# Autodesk Inventor assembly: Drivetrain Side
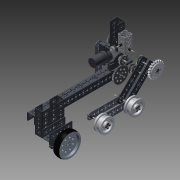
[picture p0: Inventor's stored thumbnail of the model, 180x180]
Saved by Autodesk Inventor 2015 (Build 190159000, 159)
## iProperties
Created: 2015-09-28
Part Number: Drivetrain Side
Document SubType Name: Assembly
Designer: Jing-Chen
Author: Jing-Chen
## Documents named in this file (25)
- C:\Users\Jing-Chen\Desktop\Bionic Hybrids 2016\Bionic-Hybrids\CAD\Drivetrain\Sub-Assemblies\Drivetrain Side.iam
- C:\Users\Jing-Chen\Desktop\Bionic Hybrids 2016\Bionic-Hybrids\Stock\Bracket-U25 - 739069.ipt
- C:\Users\Jing-Chen\Desktop\Bionic Hybrids 2016\Bionic-Hybrids\CAD\Drivetrain\Sub-Assemblies\Wheel Assembly.iam
- C:\Users\Jing-Chen\Desktop\Bionic Hybrids 2016\Bionic-Hybrids\CAD\Drivetrain\Sub-Assemblies\Track Frame Assembly.iam
- C:\Users\Jing-Chen\Desktop\Bionic Hybrids 2016\Bionic-Hybrids\Stock\Bearing-Thrust - 739091.ipt
- C:\Users\Jing-Chen\Desktop\Bionic Hybrids 2016\Bionic-Hybrids\Stock\Motor Mount - 739089.ipt
- C:\Users\Jing-Chen\Desktop\Bionic Hybrids 2016\Bionic-Hybrids\Stock\Bracket-U5 - 739066.ipt
- C:\Users\Jing-Chen\Desktop\Bionic Hybrids 2016\Bionic-Hybrids\CAD\General\Modified Parts\Movable Motor.iam
- C:\Users\Jing-Chen\Desktop\Bionic Hybrids 2016\Bionic-Hybrids\Stock\Gear-80 tooth - 731901.ipt
- C:\Users\Jing-Chen\Desktop\Bionic Hybrids 2016\Bionic-Hybrids\Stock\Plate-2x1 Long - 739061.ipt
- C:\Users\Jing-Chen\Desktop\Bionic Hybrids 2016\Bionic-Hybrids\Stock\Shaft Collar-Setscrew, Axle, Mountable - 739079.iam
- C:\Users\Jing-Chen\Desktop\Bionic Hybrids 2016\Bionic-Hybrids\Stock\Screw 0.5in - 739097.ipt
- C:\Users\Jing-Chen\Desktop\Bionic Hybrids 2016\Bionic-Hybrids\Stock\Shaft Collar-Setscrew, Axle, Mountable - 739172.iam
- C:\Users\Jing-Chen\Desktop\Bionic Hybrids 2016\Bionic-Hybrids\Stock\Gear-40 tooth - 731901.ipt
- C:\Users\Jing-Chen\Desktop\Bionic Hybrids 2016\Bionic-Hybrids\Stock\Nut-Locking - 739094.ipt
- C:\Users\Jing-Chen\Desktop\Bionic Hybrids 2016\Bionic-Hybrids\CAD\General\40-tooth Gear Assembly.iam
- C:\Users\Jing-Chen\Desktop\Bionic Hybrids 2016\Bionic-Hybrids\Stock\Plate-9x1 - 739272.ipt
- C:\Users\Jing-Chen\Desktop\Bionic Hybrids 2016\Bionic-Hybrids\New Stock\Worm Gear Abstract.iam
- C:\Users\Jing-Chen\Desktop\Bionic Hybrids 2016\Bionic-Hybrids\Stock\Shaft Collar-Setscrew, Axle - 739092.iam
- C:\Users\Jing-Chen\Desktop\Bionic Hybrids 2016\Bionic-Hybrids\CAD\General\Modified Parts\55mm axle.ipt
- C:\Users\Jing-Chen\Desktop\Bionic Hybrids 2016\Bionic-Hybrids\Stock\Axle-100mm - 739088.ipt
- C:\Users\Jing-Chen\Desktop\Bionic Hybrids 2016\Bionic-Hybrids\CAD\General\Modified Parts\Cut 100mm axle.ipt
- C:\Users\Jing-Chen\Desktop\Bionic Hybrids 2016\Bionic-Hybrids\Stock\Screw 1.5in - 739195.ipt
- C:\Users\Jing-Chen\Desktop\Bionic Hybrids 2016\Bionic-Hybrids\Stock\Bracket-U9 - 739067.ipt
- C:\Users\Jing-Chen\Desktop\Bionic Hybrids 2016\Bionic-Hybrids\CAD\Drivetrain\Sub-Assemblies\Track Frame Assembly with Side Guards.iam
## Components (77 placed, 24 different names)
1. Track Frame Assembly:1 [sub-assembly] — Mate:33, Mate:36, Rotation:2, Mate:157, Mate:160, Angle:11, Mate:258, Mate:259, Flush:11
2. Bearing-Thrust - 739091:1 — Mate:33, Mate:36, Mate:60, Mate:61
3. Motor Mount - 739089:1 — Mate:40, Flush:1, Mate:51, Mate:52, Mate:53, Mate:234, Mate:235, Mate:236, Mate:237
4. Wheel Assembly:1 [sub-assembly] — Angle:2, Mate:41, Flush:2
5. Movable Motor:1 [sub-assembly] — Mate:40, Flush:1, Angle:1, Angle:2, Mate:41, Flush:2
6. Bracket-U5 - 739066:1 — Mate:44, Mate:46, Mate:47, Mate:51, Mate:52, Mate:53, Mate:248, Mate:249
7. Bracket-U5 - 739066:2 — Mate:44, Mate:46, Mate:47, Mate:54, Mate:55, Mate:56
8. Bracket-U5 - 739066:3 — Mate:57, Mate:58, Mate:59
9. Bracket-U25 - 739069:1 — Mate:54, Mate:55, Mate:56, Mate:57, Mate:58, Mate:59, Mate:60, Mate:61, Mate:62, Angle:3, Mate:81, Mate:96, Mate:97, Mate:126, Mate:128, Mate:130, Mate:131, Mate:132, Mate:133, Mate:135, Mate:137, Mate:140, Mate:141, Mate:165, Mate:170, Mate:173, Mate:198, Mate:204, Mate:212, Mate:230, Mate:233
10. Movable Motor:2 [sub-assembly] — Mate:64, Flush:3, Angle:4, Angle:5, Mate:108
11. Motor Mount - 739089:2 — Mate:62, Angle:3, Mate:64, Flush:3, Mate:82, Mate:83, Mate:116, Mate:199, Mate:200, Mate:202, Mate:203
12. Plate-2x1 Long - 739061:2 — Mate:81, Mate:82, Mate:83, Mate:116
13. Shaft Collar-Setscrew, Axle, Mountable - 739079:1 [sub-assembly] — Angle:5, Mate:104, Mate:105, Mate:106, Mate:107, Mate:108, Mate:109, Mate:111
14. Screw 0.5in - 739097:1 — Mate:105, Mate:110, Mate:113
15. Screw 0.5in - 739097:2 — Mate:107, Mate:112
16. Screw 0.5in - 739097:3 — Mate:104, Mate:114
17. Screw 0.5in - 739097:4 — Mate:106, Mate:115
18. Bearing-Thrust - 739091:2 — Mate:96, Mate:97, Mate:100
19. Shaft Collar-Setscrew, Axle, Mountable - 739172:1 [sub-assembly] — Mate:100, Mate:102, Mate:103, Mate:121, Mate:122, Mate:123, Mate:124, Mate:179
20. Gear-80 tooth - 731901:2 — Mate:102, Mate:103, Flush:4, Rotation:1, Rotation:2, Mate:117, Mate:118, Mate:119, Mate:120, Mate:178, Flush:7
21. Gear-40 tooth - 731901:1 — Mate:109, Mate:110, Mate:111, Mate:112, Mate:113, Mate:114, Mate:115, Flush:4, Rotation:1
22. Screw 0.5in - 739097:5 — Mate:118, Mate:122
23. Screw 0.5in - 739097:6 — Mate:117, Mate:121
24. Screw 0.5in - 739097:7 — Mate:119, Mate:123
25. Screw 0.5in - 739097:8 — Mate:120, Mate:124, Mate:178
26. Bearing-Thrust - 739091:3 — Mate:126, Mate:128, Mate:177, Mate:181
27. Screw 0.5in - 739097:9 — Mate:133, Mate:134, Mate:207, Mate:208
28. Screw 0.5in - 739097:10 — Mate:131, Mate:136, Mate:206, Mate:209
29. Screw 0.5in - 739097:11 — Mate:130, Mate:139, Mate:210
30. Screw 0.5in - 739097:12 — Mate:132, Mate:138, Mate:211
31. Nut-Locking - 739094:1 — Mate:136, Mate:137
32. Nut-Locking - 739094:2 — Mate:134, Mate:135
33. Nut-Locking - 739094:3 — Mate:139, Mate:140
34. Nut-Locking - 739094:4 — Mate:138, Mate:141
35. Bearing-Thrust - 739091:4 — Mate:158, Mate:160, Mate:221
36. Bearing-Thrust - 739091:5 — Mate:182, Mate:184, Mate:219, Mate:220
37. Bearing-Thrust - 739091:6 — Mate:187, Mate:189, Mate:215, Mate:216
38. Bearing-Thrust - 739091:7 — Mate:186, Mate:217, Mate:218
39. 40-tooth Gear Assembly:1 [sub-assembly] — Mate:157, Mate:158, Angle:11, Rotation:4
40. 40-tooth Gear Assembly:2 [sub-assembly] — Mate:183, Mate:184, Flush:8, Rotation:3, Rotation:4
41. 40-tooth Gear Assembly:3 [sub-assembly] — Mate:188, Mate:189, Flush:9, Rotation:3, Angle:14
42. Movable Motor:3 [sub-assembly] — Mate:169, Flush:6, Angle:7, Angle:12, Mate:191, Flush:10, Mate:192
43. Motor Mount - 739089:3 — Mate:169, Flush:6, Mate:171, Angle:10, Mate:172, Mate:238, Mate:239, Mate:240, Mate:241
44. Plate-9x1 - 739272:1 — Mate:165, Mate:170, Mate:171, Angle:10, Mate:172, Mate:173, Mate:226, Mate:227, Mate:228, Mate:229, Mate:243, Mate:247
45. Worm Gearbox, Ratio 20:1 [sub-assembly] — Mate:190, Mate:213, Mate:214, Mate:224
46. 55mm axle:1 — Mate:177, Mate:179, Flush:7, Mate:180
47. Shaft Collar-Setscrew, Axle - 739092:1 [sub-assembly] — Mate:180, Mate:181
48. Shaft Collar-Setscrew, Axle - 739092:2 [sub-assembly] — Mate:185, Mate:186
49. 55mm axle:2 — Mate:182, Mate:183, Flush:8, Mate:185
50. Axle-100mm - 739088:1 — Mate:187, Mate:188, Flush:9, Rotation:5, Angle:14, Mate:214
51. Shaft Collar-Setscrew, Axle, Mountable - 739079:2 [sub-assembly] — Angle:12, Mate:191, Flush:10, Mate:194, Mate:195
52. Shaft Collar-Setscrew, Axle, Mountable - 739172:2 [sub-assembly] — Angle:13, Mate:193, Mate:194, Mate:195, Mate:250, Mate:251, Mate:252, Mate:253, Mate:254, Mate:255, Mate:256, Mate:257
53. Cut 100mm axle:1 — Mate:190, Mate:192, Angle:13, Mate:193, Rotation:5
54. Screw 1.5in - 739195:1 — Mate:199, Mate:200, Mate:201
55. Screw 0.5in - 739097:22 — Mate:222, Mate:223, Mate:225
56. Screw 0.5in - 739097:23 — Mate:227, Mate:229, Mate:232
57. Nut-Locking - 739094:5 — Mate:223, Mate:224
58. Nut-Locking - 739094:6 — Mate:230, Mate:231
59. Nut-Locking - 739094:7 — Mate:198, Mate:201
60. Nut-Locking - 739094:8 — Mate:204, Mate:205
61. Screw 0.5in - 739097:24 — Mate:226, Mate:228, Mate:231
62. Screw 1.5in - 739195:2 — Mate:202, Mate:203, Mate:205
63. Bracket-U9 - 739067:1 — Mate:206, Mate:207, Mate:208, Mate:209, Mate:210, Mate:211, Mate:212, Mate:213, Mate:215, Mate:216, Mate:217, Mate:218, Mate:219, Mate:220, Mate:221, Mate:222, Mate:225
64. Nut-Locking - 739094:9 — Mate:232, Mate:233
65. Screw 1.5in - 739195:3 — Mate:236, Mate:237, Mate:244
66. Screw 1.5in - 739195:4 — Mate:238, Mate:239, Mate:242
67. Screw 1.5in - 739195:5 — Mate:234, Mate:235, Mate:245
68. Screw 1.5in - 739195:6 — Mate:240, Mate:241, Mate:246
69. Nut-Locking - 739094:10 — Mate:242, Mate:243
70. Nut-Locking - 739094:11 — Mate:244, Mate:249
71. Nut-Locking - 739094:12 — Mate:245, Mate:248
72. Nut-Locking - 739094:13 — Mate:246, Mate:247
73. Screw 0.5in - 739097:25 — Mate:255, Mate:257
74. Screw 0.5in - 739097:26 — Mate:254, Mate:256
75. Screw 0.5in - 739097:27 — Mate:251, Mate:252
76. Screw 0.5in - 739097:28 — Mate:250, Mate:253
77. Track Frame Assembly with Side Guards:1 [sub-assembly] — Mate:258, Mate:259, Flush:11
## Relationships (179: Mate 153, Angle 11, Flush 10, RelateRotation 5)
- Mate:33: Track Frame Assembly:1 ↔ Bearing-Thrust - 739091:1
- Mate:36: Track Frame Assembly:1 ↔ Bearing-Thrust - 739091:1
- Mate:40: Motor Mount - 739089:1 ↔ Movable Motor:1
- Flush:1: Motor Mount - 739089:1 ↔ Movable Motor:1
- Angle:1 (180 deg): Movable Motor:1
- Angle:2 (180 deg): Wheel Assembly:1 ↔ Movable Motor:1
- Mate:41: Wheel Assembly:1 ↔ Movable Motor:1
- Flush:2: Wheel Assembly:1 ↔ Movable Motor:1
- Mate:44: Bracket-U5 - 739066:1 ↔ Bracket-U5 - 739066:2
- Mate:46: Bracket-U5 - 739066:1 ↔ Bracket-U5 - 739066:2
- Mate:47: Bracket-U5 - 739066:1 ↔ Bracket-U5 - 739066:2
- Mate:51: Motor Mount - 739089:1 ↔ Bracket-U5 - 739066:1
- Mate:52: Motor Mount - 739089:1 ↔ Bracket-U5 - 739066:1
- Mate:53: Motor Mount - 739089:1 ↔ Bracket-U5 - 739066:1
- Mate:54: Bracket-U5 - 739066:2 ↔ Bracket-U25 - 739069:1
- Mate:55: Bracket-U5 - 739066:2 ↔ Bracket-U25 - 739069:1
- Mate:56: Bracket-U5 - 739066:2 ↔ Bracket-U25 - 739069:1
- Mate:57: Bracket-U5 - 739066:3 ↔ Bracket-U25 - 739069:1
- Mate:58: Bracket-U5 - 739066:3 ↔ Bracket-U25 - 739069:1
- Mate:59: Bracket-U5 - 739066:3 ↔ Bracket-U25 - 739069:1
- Mate:60: Bearing-Thrust - 739091:1 ↔ Bracket-U25 - 739069:1
- Mate:61: Bearing-Thrust - 739091:1 ↔ Bracket-U25 - 739069:1
- Mate:62: Bracket-U25 - 739069:1 ↔ Motor Mount - 739089:2
- Angle:3 (0 deg): Bracket-U25 - 739069:1 ↔ Motor Mount - 739089:2
- Mate:64: Movable Motor:2 ↔ Motor Mount - 739089:2
- Flush:3: Movable Motor:2 ↔ Motor Mount - 739089:2
- Angle:4 (190 deg): Movable Motor:2
- Mate:81: Bracket-U25 - 739069:1 ↔ Plate-2x1 Long - 739061:2
- Mate:82: Motor Mount - 739089:2 ↔ Plate-2x1 Long - 739061:2
- Mate:83: Motor Mount - 739089:2 ↔ Plate-2x1 Long - 739061:2
- Angle:5 (180 deg): Movable Motor:2 ↔ Shaft Collar-Setscrew, Axle, Mountable - 739079:1
- Mate:96: Bracket-U25 - 739069:1 ↔ Bearing-Thrust - 739091:2
- Mate:97: Bracket-U25 - 739069:1 ↔ Bearing-Thrust - 739091:2
- Mate:100: Bearing-Thrust - 739091:2 ↔ Shaft Collar-Setscrew, Axle, Mountable - 739172:1
- Mate:102: Shaft Collar-Setscrew, Axle, Mountable - 739172:1 ↔ Gear-80 tooth - 731901:2
- Mate:103: Shaft Collar-Setscrew, Axle, Mountable - 739172:1 ↔ Gear-80 tooth - 731901:2
- Mate:104: Shaft Collar-Setscrew, Axle, Mountable - 739079:1 ↔ Screw 0.5in - 739097:3
- Mate:105: Shaft Collar-Setscrew, Axle, Mountable - 739079:1 ↔ Screw 0.5in - 739097:1
- Mate:106: Shaft Collar-Setscrew, Axle, Mountable - 739079:1 ↔ Screw 0.5in - 739097:4
- Mate:107: Shaft Collar-Setscrew, Axle, Mountable - 739079:1 ↔ Screw 0.5in - 739097:2
- Mate:108: Movable Motor:2 ↔ Shaft Collar-Setscrew, Axle, Mountable - 739079:1
- Mate:109: Shaft Collar-Setscrew, Axle, Mountable - 739079:1 ↔ Gear-40 tooth - 731901:1
- Mate:110: Screw 0.5in - 739097:1 ↔ Gear-40 tooth - 731901:1
- Mate:111: Shaft Collar-Setscrew, Axle, Mountable - 739079:1 ↔ Gear-40 tooth - 731901:1
- Mate:112: Screw 0.5in - 739097:2 ↔ Gear-40 tooth - 731901:1
- Mate:113: Screw 0.5in - 739097:1 ↔ Gear-40 tooth - 731901:1
- Mate:114: Screw 0.5in - 739097:3 ↔ Gear-40 tooth - 731901:1
- Mate:115: Screw 0.5in - 739097:4 ↔ Gear-40 tooth - 731901:1
- Mate:116: Motor Mount - 739089:2 ↔ Plate-2x1 Long - 739061:2
- Flush:4: Gear-80 tooth - 731901:2 ↔ Gear-40 tooth - 731901:1
- Rotation:1 [RelateRotation] (0.5 ul): Gear-80 tooth - 731901:2 ↔ Gear-40 tooth - 731901:1
- Rotation:2 [RelateRotation] (2 ul): Track Frame Assembly:1 ↔ Gear-80 tooth - 731901:2
- Mate:117: Gear-80 tooth - 731901:2 ↔ Screw 0.5in - 739097:6
- Mate:118: Gear-80 tooth - 731901:2 ↔ Screw 0.5in - 739097:5
- Mate:119: Gear-80 tooth - 731901:2 ↔ Screw 0.5in - 739097:7
- Mate:120: Gear-80 tooth - 731901:2 ↔ Screw 0.5in - 739097:8
- Mate:121: Shaft Collar-Setscrew, Axle, Mountable - 739172:1 ↔ Screw 0.5in - 739097:6
- Mate:122: Shaft Collar-Setscrew, Axle, Mountable - 739172:1 ↔ Screw 0.5in - 739097:5
- Mate:123: Shaft Collar-Setscrew, Axle, Mountable - 739172:1 ↔ Screw 0.5in - 739097:7
- Mate:124: Shaft Collar-Setscrew, Axle, Mountable - 739172:1 ↔ Screw 0.5in - 739097:8
- Mate:126: Bracket-U25 - 739069:1 ↔ Bearing-Thrust - 739091:3
- Mate:128: Bracket-U25 - 739069:1 ↔ Bearing-Thrust - 739091:3
- Mate:130: Bracket-U25 - 739069:1 ↔ Screw 0.5in - 739097:11
- Mate:131: Bracket-U25 - 739069:1 ↔ Screw 0.5in - 739097:10
- Mate:132: Bracket-U25 - 739069:1 ↔ Screw 0.5in - 739097:12
- Mate:133: Bracket-U25 - 739069:1 ↔ Screw 0.5in - 739097:9
- Mate:134: Screw 0.5in - 739097:9 ↔ Nut-Locking - 739094:2
- Mate:135: Bracket-U25 - 739069:1 ↔ Nut-Locking - 739094:2
- Mate:136: Screw 0.5in - 739097:10 ↔ Nut-Locking - 739094:1
- Mate:137: Bracket-U25 - 739069:1 ↔ Nut-Locking - 739094:1
- Mate:138: Screw 0.5in - 739097:12 ↔ Nut-Locking - 739094:4
- Mate:139: Screw 0.5in - 739097:11 ↔ Nut-Locking - 739094:3
- Mate:140: Bracket-U25 - 739069:1 ↔ Nut-Locking - 739094:3
- Mate:141: Bracket-U25 - 739069:1 ↔ Nut-Locking - 739094:4
- Mate:157: Track Frame Assembly:1 ↔ 40-tooth Gear Assembly:1
- Mate:158: Bearing-Thrust - 739091:4 ↔ 40-tooth Gear Assembly:1
- Mate:160: Track Frame Assembly:1 ↔ Bearing-Thrust - 739091:4
- Mate:165: Bracket-U25 - 739069:1 ↔ Plate-9x1 - 739272:1
- Mate:169: Movable Motor:3 ↔ Motor Mount - 739089:3
- Flush:6: Movable Motor:3 ↔ Motor Mount - 739089:3
- Angle:7 (180 deg): Movable Motor:3
- Mate:170: Bracket-U25 - 739069:1 ↔ Plate-9x1 - 739272:1
- Mate:171: Motor Mount - 739089:3 ↔ Plate-9x1 - 739272:1
- Angle:10 (180 deg): Motor Mount - 739089:3 ↔ Plate-9x1 - 739272:1
- Mate:172: Motor Mount - 739089:3 ↔ Plate-9x1 - 739272:1
- Mate:173: Bracket-U25 - 739069:1 ↔ Plate-9x1 - 739272:1
- Mate:177: Bearing-Thrust - 739091:3 ↔ 55mm axle:1
- Mate:178: Gear-80 tooth - 731901:2 ↔ Screw 0.5in - 739097:8
- Mate:179: Shaft Collar-Setscrew, Axle, Mountable - 739172:1 ↔ 55mm axle:1
- Flush:7: Gear-80 tooth - 731901:2 ↔ 55mm axle:1
- Mate:180: 55mm axle:1 ↔ Shaft Collar-Setscrew, Axle - 739092:1
- Mate:181: Bearing-Thrust - 739091:3 ↔ Shaft Collar-Setscrew, Axle - 739092:1
- Mate:182: Bearing-Thrust - 739091:5 ↔ 55mm axle:2
- Mate:183: 40-tooth Gear Assembly:2 ↔ 55mm axle:2
- Mate:184: Bearing-Thrust - 739091:5 ↔ 40-tooth Gear Assembly:2
- Flush:8: 40-tooth Gear Assembly:2 ↔ 55mm axle:2
- Angle:11 (180 deg): Track Frame Assembly:1 ↔ 40-tooth Gear Assembly:1
- Mate:185: Shaft Collar-Setscrew, Axle - 739092:2 ↔ 55mm axle:2
- Mate:186: Bearing-Thrust - 739091:7 ↔ Shaft Collar-Setscrew, Axle - 739092:2
- Mate:187: Bearing-Thrust - 739091:6 ↔ Axle-100mm - 739088:1
- Mate:188: 40-tooth Gear Assembly:3 ↔ Axle-100mm - 739088:1
- Mate:189: Bearing-Thrust - 739091:6 ↔ 40-tooth Gear Assembly:3
- Flush:9: 40-tooth Gear Assembly:3 ↔ Axle-100mm - 739088:1
- Rotation:3 [RelateRotation] (1 ul): 40-tooth Gear Assembly:2 ↔ 40-tooth Gear Assembly:3
- Rotation:4 [RelateRotation] (1 ul): 40-tooth Gear Assembly:1 ↔ 40-tooth Gear Assembly:2
- Mate:190: Worm Gearbox, Ratio 20:1 ↔ Cut 100mm axle:1
- Angle:12 (180 deg): Movable Motor:3 ↔ Shaft Collar-Setscrew, Axle, Mountable - 739079:2
- Mate:191: Movable Motor:3 ↔ Shaft Collar-Setscrew, Axle, Mountable - 739079:2
- Flush:10: Movable Motor:3 ↔ Shaft Collar-Setscrew, Axle, Mountable - 739079:2
- Mate:192: Movable Motor:3 ↔ Cut 100mm axle:1
- Angle:13 (180 deg): Shaft Collar-Setscrew, Axle, Mountable - 739172:2 ↔ Cut 100mm axle:1
- Mate:193: Shaft Collar-Setscrew, Axle, Mountable - 739172:2 ↔ Cut 100mm axle:1
- Mate:194: Shaft Collar-Setscrew, Axle, Mountable - 739079:2 ↔ Shaft Collar-Setscrew, Axle, Mountable - 739172:2
- Mate:195: Shaft Collar-Setscrew, Axle, Mountable - 739079:2 ↔ Shaft Collar-Setscrew, Axle, Mountable - 739172:2
- Rotation:5 [RelateRotation] (0.05 ul): Axle-100mm - 739088:1 ↔ Cut 100mm axle:1
- Angle:14 (180 deg): 40-tooth Gear Assembly:3 ↔ Axle-100mm - 739088:1
- Mate:198: Bracket-U25 - 739069:1 ↔ Nut-Locking - 739094:7
- Mate:199: Motor Mount - 739089:2 ↔ Screw 1.5in - 739195:1
- Mate:200: Motor Mount - 739089:2 ↔ Screw 1.5in - 739195:1
- Mate:201: Screw 1.5in - 739195:1 ↔ Nut-Locking - 739094:7
- Mate:202: Motor Mount - 739089:2 ↔ Screw 1.5in - 739195:2
- Mate:203: Motor Mount - 739089:2 ↔ Screw 1.5in - 739195:2
- Mate:204: Bracket-U25 - 739069:1 ↔ Nut-Locking - 739094:8
- Mate:205: Nut-Locking - 739094:8 ↔ Screw 1.5in - 739195:2
- Mate:206: Screw 0.5in - 739097:10 ↔ Bracket-U9 - 739067:1
- Mate:207: Screw 0.5in - 739097:9 ↔ Bracket-U9 - 739067:1
- Mate:208: Screw 0.5in - 739097:9 ↔ Bracket-U9 - 739067:1
- Mate:209: Screw 0.5in - 739097:10 ↔ Bracket-U9 - 739067:1
- Mate:210: Screw 0.5in - 739097:11 ↔ Bracket-U9 - 739067:1
- Mate:211: Screw 0.5in - 739097:12 ↔ Bracket-U9 - 739067:1
- Mate:212: Bracket-U25 - 739069:1 ↔ Bracket-U9 - 739067:1
- Mate:213: Worm Gearbox, Ratio 20:1 ↔ Bracket-U9 - 739067:1
- Mate:214: Worm Gearbox, Ratio 20:1 ↔ Axle-100mm - 739088:1
- Mate:215: Bearing-Thrust - 739091:6 ↔ Bracket-U9 - 739067:1
- Mate:216: Bearing-Thrust - 739091:6 ↔ Bracket-U9 - 739067:1
- Mate:217: Bearing-Thrust - 739091:7 ↔ Bracket-U9 - 739067:1
- Mate:218: Bearing-Thrust - 739091:7 ↔ Bracket-U9 - 739067:1
- Mate:219: Bearing-Thrust - 739091:5 ↔ Bracket-U9 - 739067:1
- Mate:220: Bearing-Thrust - 739091:5 ↔ Bracket-U9 - 739067:1
- Mate:221: Bearing-Thrust - 739091:4 ↔ Bracket-U9 - 739067:1
- Mate:222: Screw 0.5in - 739097:22 ↔ Bracket-U9 - 739067:1
- Mate:223: Screw 0.5in - 739097:22 ↔ Nut-Locking - 739094:5
- Mate:224: Worm Gearbox, Ratio 20:1 ↔ Nut-Locking - 739094:5
- Mate:225: Screw 0.5in - 739097:22 ↔ Bracket-U9 - 739067:1
- Mate:226: Plate-9x1 - 739272:1 ↔ Screw 0.5in - 739097:24
- Mate:227: Plate-9x1 - 739272:1 ↔ Screw 0.5in - 739097:23
- Mate:228: Plate-9x1 - 739272:1 ↔ Screw 0.5in - 739097:24
- Mate:229: Plate-9x1 - 739272:1 ↔ Screw 0.5in - 739097:23
- Mate:230: Bracket-U25 - 739069:1 ↔ Nut-Locking - 739094:6
- Mate:231: Nut-Locking - 739094:6 ↔ Screw 0.5in - 739097:24
- Mate:232: Screw 0.5in - 739097:23 ↔ Nut-Locking - 739094:9
- Mate:233: Bracket-U25 - 739069:1 ↔ Nut-Locking - 739094:9
- Mate:234: Motor Mount - 739089:1 ↔ Screw 1.5in - 739195:5
- Mate:235: Motor Mount - 739089:1 ↔ Screw 1.5in - 739195:5
- Mate:236: Motor Mount - 739089:1 ↔ Screw 1.5in - 739195:3
- Mate:237: Motor Mount - 739089:1 ↔ Screw 1.5in - 739195:3
- Mate:238: Motor Mount - 739089:3 ↔ Screw 1.5in - 739195:4
- Mate:239: Motor Mount - 739089:3 ↔ Screw 1.5in - 739195:4
- Mate:240: Motor Mount - 739089:3 ↔ Screw 1.5in - 739195:6
- Mate:241: Motor Mount - 739089:3 ↔ Screw 1.5in - 739195:6
- Mate:242: Screw 1.5in - 739195:4 ↔ Nut-Locking - 739094:10
- Mate:243: Plate-9x1 - 739272:1 ↔ Nut-Locking - 739094:10
- Mate:244: Screw 1.5in - 739195:3 ↔ Nut-Locking - 739094:11
- Mate:245: Screw 1.5in - 739195:5 ↔ Nut-Locking - 739094:12
- Mate:246: Screw 1.5in - 739195:6 ↔ Nut-Locking - 739094:13
- Mate:247: Plate-9x1 - 739272:1 ↔ Nut-Locking - 739094:13
- Mate:248: Bracket-U5 - 739066:1 ↔ Nut-Locking - 739094:12
- Mate:249: Bracket-U5 - 739066:1 ↔ Nut-Locking - 739094:11
- Mate:250: Shaft Collar-Setscrew, Axle, Mountable - 739172:2 ↔ Screw 0.5in - 739097:28
- Mate:251: Shaft Collar-Setscrew, Axle, Mountable - 739172:2 ↔ Screw 0.5in - 739097:27
- Mate:252: Shaft Collar-Setscrew, Axle, Mountable - 739172:2 ↔ Screw 0.5in - 739097:27
- Mate:253: Shaft Collar-Setscrew, Axle, Mountable - 739172:2 ↔ Screw 0.5in - 739097:28
- Mate:254: Shaft Collar-Setscrew, Axle, Mountable - 739172:2 ↔ Screw 0.5in - 739097:26
- Mate:255: Shaft Collar-Setscrew, Axle, Mountable - 739172:2 ↔ Screw 0.5in - 739097:25
- Mate:256: Shaft Collar-Setscrew, Axle, Mountable - 739172:2 ↔ Screw 0.5in - 739097:26
- Mate:257: Shaft Collar-Setscrew, Axle, Mountable - 739172:2 ↔ Screw 0.5in - 739097:25
- Mate:258: Track Frame Assembly:1 ↔ Track Frame Assembly with Side Guards:1
- Mate:259: Track Frame Assembly:1 ↔ Track Frame Assembly with Side Guards:1
- Flush:11: Track Frame Assembly:1 ↔ Track Frame Assembly with Side Guards:1
